# Autodesk Inventor assembly: DoubleSolenoidRack
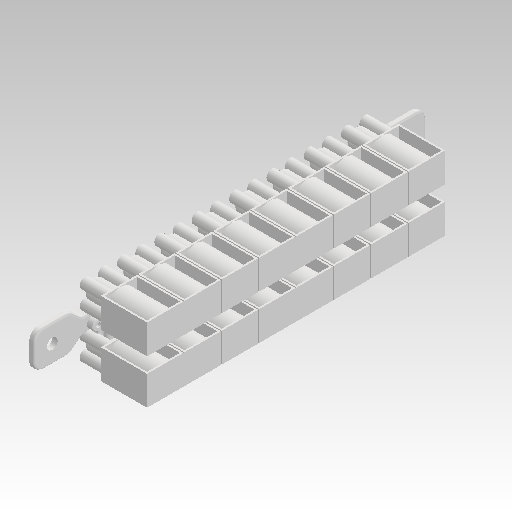
[picture p0: Inventor's stored thumbnail of the model, 512x512]
Saved by Autodesk Inventor 2020 (Build 240168000, 168)
## iProperties
Created: 2021-09-21
Part Number: DoubleSolenoidRack
Document SubType Name: Assembly
Designer: DDeGo
Author: DDeGo
## Documents named in this file (4)
- C:\Users\DDeGo\Documents\Drew\Projects\Gravity-Holo-Display\cad\DoubleSolenoidRack.iam
- C:\Users\DDeGo\Documents\Drew\Projects\Gravity-Holo-Display\cad\DoubleSolenoidBracket.ipt
- C:\Users\DDeGo\Documents\Drew\Projects\Gravity-Holo-Display\cad\DoubleSolenoidHead.ipt
- C:\Users\DDeGo\Documents\Drew\Projects\Gravity-Holo-Display\cad\Solenoid.ipt
## Components (25 placed, 3 different names)
1. DoubleSolenoidBracket:1 — Mate:1, Mate:2, Mate:3, Angle:1
2. DoubleSolenoidHead:1 — Mate:1, Mate:2, Mate:3, Mate:4, Mate:5, Mate:6, Mate:7
3. Solenoid:2 — Mate:4, Mate:6, Angle:2
4. Solenoid:1 — Mate:5, Mate:7, Angle:1, Angle:2
5. DoubleSolenoidHead:2
6. Solenoid:3
7. Solenoid:4
8. DoubleSolenoidHead:3
9. Solenoid:5
10. Solenoid:6
11. DoubleSolenoidHead:4
12. Solenoid:7
13. Solenoid:8
14. DoubleSolenoidHead:5
15. Solenoid:9
16. Solenoid:10
17. DoubleSolenoidHead:6
18. Solenoid:11
19. Solenoid:12
20. DoubleSolenoidHead:7
21. Solenoid:13
22. Solenoid:14
23. DoubleSolenoidHead:8
24. Solenoid:15
25. Solenoid:16
## Component patterns: (8 elements, first: DoubleSolenoidHead:1 + Solenoid:2 + Solenoid:1)
## Relationships (9: Mate 7, Angle 2)
- Mate:1: DoubleSolenoidBracket:1 ↔ DoubleSolenoidHead:1
- Mate:2: DoubleSolenoidBracket:1 ↔ DoubleSolenoidHead:1
- Mate:3: DoubleSolenoidBracket:1 ↔ DoubleSolenoidHead:1
- Mate:4: DoubleSolenoidHead:1 ↔ Solenoid:2
- Mate:5: DoubleSolenoidHead:1 ↔ Solenoid:1
- Mate:6: DoubleSolenoidHead:1 ↔ Solenoid:2
- Mate:7: DoubleSolenoidHead:1 ↔ Solenoid:1
- Angle:1 (0 deg): DoubleSolenoidBracket:1 ↔ Solenoid:1
- Angle:2 (0 deg): Solenoid:2 ↔ Solenoid:1
